# Autodesk Inventor assembly: CycloidalDrive2
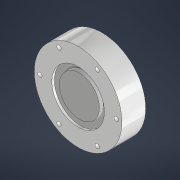
[picture p0: Inventor's stored thumbnail of the model, 180x180]
Saved by Autodesk Inventor 2021 (Build 250183000, 183)
## iProperties
Created: 2022-10-07
Part Number: CycloidalDrive2
Document SubType Name: Assembly
Designer: MicnedSQ
Author: MicnedSQ
## Documents named in this file (4)
- C:\Users\MicnedSQ\Desktop\V1\RotatingBase\CycloidalDrive\CycloidalDrive2.iam
- C:\Users\MicnedSQ\Desktop\V1\RotatingBase\CycloidalDrive\Bottom.ipt
- C:\Users\MicnedSQ\Desktop\V1\RotatingBase\CycloidalDrive\OutputShaft.ipt
- C:\Users\MicnedSQ\Desktop\V1\RotatingBase\CycloidalDrive\CycloidalDisc.ipt
## Components (3 placed, 3 different names)
1. Bottom:1 — Obrotowe:1
2. OutputShaft:1 — Obrotowe:1, Obrotowe:2, Obrót:1
3. CycloidalDisc:1 — Obrotowe:2, Obrót:1
## Relationships (3: RevoluteJoint 2, RelateRotation 1)
- Obrotowe:1 [RevoluteJoint]: Bottom:1 ↔ OutputShaft:1
- Obrotowe:2 [RevoluteJoint]: OutputShaft:1 ↔ CycloidalDisc:1
- Obrót:1 [RelateRotation] (0.0435 ul): OutputShaft:1 ↔ CycloidalDisc:1
